# Autodesk Inventor assembly: 正齿轮
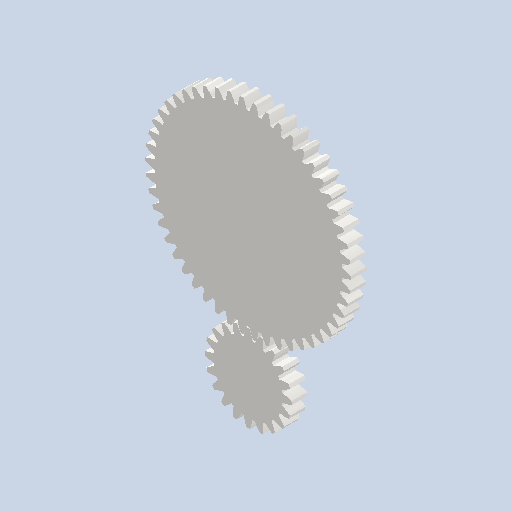
[picture p0: Inventor's stored thumbnail of the model, 512x512]
Saved by Autodesk Inventor 2022 (Build 260153000, 153)
## iProperties
ClientObjectVersion: 1
Created: 2023-02-21
Part Number: 正齿轮
Document SubType Name: Assembly
Designer: 李承轩
Categories: <?xml version="1.0" encoding="UTF-16"?> <MemberInstance><Categories><FamilyTemplate/><ParamToTemplateMap><ParamToTemplate><ParamToTemplate CategoryParameter="//CategoryParameter[@InternalName='9E91F9C2-1A37-4abf-91CE-B4CF7EE75BC6']" ConstantValue="10000000.000000"/></ParamToTemplate><ParamToTemplate><ParamToTemplate CategoryParameter="//CategoryParameter[@InternalName='2AFF4D85-1BD8-4ea8-8D18-96A2CAB0895B']" ConstantValue="9800000.000000"/></ParamToTemplate><ParamToTemplate><ParamToTemplate CategoryParameter="//CategoryParameter[@InternalName='E8E51088-10FD-40b5-B945-790B32C7EFBA']" ConstantValue="104.719755"/></ParamToTemplate><ParamToTemplate><ParamToTemplate CategoryParameter="//CategoryParameter[@InternalName='752D88A1-A866-440c-81C2-59259440B19C']" ConstantValue="41.887902"/></ParamToTemplate><ParamToTemplate><ParamToTemplate CategoryParameter="//CategoryParameter[@InternalName='5F43FD89-24D7-49f6-B63B-C3D8E39D8A69']" ConstantValue="95492.965855"/></ParamToTemplate><ParamToTemplate><ParamToTemplate CategoryParameter="//CategoryParameter[@InternalName='8D239626-6A17-497c-A9EF-C1C80B41D68F']" ConstantValue="233957.766345"/></ParamToTemplate><ParamToTemplate><ParamToTemplate CategoryParameter="//CategoryParameter[@InternalName='41D48E04-51D6-4192-AEE3-C42B8672B6EA']" ConstantValue="0.980000"/></ParamToTemplate><ParamToTemplate><ParamToTemplate CategoryParameter="//CategoryParameter[@InternalName='E5FFB0D5-AABD-4279-8B19-7DCFF75B68C0']" ConstantValue="6"/></ParamToTemplate></ParamToTemplateMap><Category DisplayName="Gears" InternalName="3565AA18-AB10-415a-941E-C703DB507537" Mnemonic="Gears"><CategoryParameter DisplayName="P" InternalName="9E91F9C2-1A37-4abf-91CE-B4CF7EE75BC6" Mnemonic="P1"/><CategoryParameter DisplayName="P" InternalName="2AFF4D85-1BD8-4ea8-8D18-96A2CAB0895B" Mnemonic="P2"/><CategoryParameter DisplayName="n" InternalName="E8E51088-10FD-40b5-B945-790B32C7EFBA" Mnemonic="n1"/><CategoryParameter DisplayName="n" InternalName="752D88A1-A866-440c-81C2-59259440B19C" Mnemonic="n2"/><CategoryParameter DisplayName="T" InternalName="5F43FD89-24D7-49f6-B63B-C3D8E39D8A69" Mnemonic="Mk1"/><CategoryParameter DisplayName="T" InternalName="8D239626-6A17-497c-A9EF-C1C80B41D68F" Mnemonic="Mk2"/><CategoryParameter DisplayName="||h|" InternalName="41D48E04-51D6-4192-AEE3-C42B8672B6EA" Mnemonic="eta"/><Category DisplayName="SpurGears" InternalName="B2B51C2B-6DC6-4009-A81E-78A8221B7E56" Mnemonic="SpurGears"><CategoryParameter DisplayName="idxIT1" InternalName="E5FFB0D5-AABD-4279-8B19-7DCFF75B68C0" Mnemonic="idxIT1"/></Category></Category></Categories></MemberInstance>
Author: 李承轩
## Documents named in this file (3)
- D:\Person products\发动机模型\动力传输1\设计加速器\正齿轮3.iam
- D:\Person products\发动机模型\动力传输1\设计加速器\正齿轮13.ipt
- D:\Person products\发动机模型\动力传输1\设计加速器\正齿轮23.ipt
## Components (2 placed, 2 different names)
1. 正齿轮1:1 — 表面齐平:1, 配合:1, 转动:1
2. 正齿轮2:1 — 表面齐平:1, 配合:1, 转动:1
## Relationships (3: Flush 1, Mate 1, RelateRotation 1)
- 表面齐平:1 [Flush]: 正齿轮1:1 ↔ 正齿轮2:1
- 配合:1 [Mate] (175 mm): 正齿轮1:1 ↔ 正齿轮2:1
- 转动:1 [RelateRotation] (0.4 ul): 正齿轮1:1 ↔ 正齿轮2:1
